# Autodesk Inventor assembly: skjellett
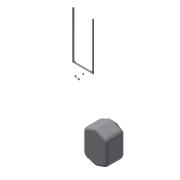
[picture p0: Inventor's stored thumbnail of the model, 180x180]
Saved by Autodesk Inventor 2014 SP1 (Build 180222100, 222)
## iProperties
Created: 2015-02-04
Part Number: skjellett
Document SubType Name: Assembly
Designer: Simen
Author: Simen
## Documents named in this file (5)
- C:\Users\Simen\Documents\git\Eit\skjellet\skjellett.iam
- main.iam
- C:\Users\Simen\Documents\git\Eit\skjellet\base.iam
- C:\Users\Simen\Documents\git\Eit\skjellet\skellett.iam
- C:\Users\Simen\Documents\git\Eit\skjellet\mount_holes_plate.ipt
## Components (3 placed, 3 different names)
1. skellett:1 [sub-assembly]
2. base:1 [sub-assembly] — Flush:1, Mate:1, Mate:2
3. mount_holes_plate:1 — Flush:1, Mate:1, Mate:2
## Relationships (3: Mate 2, Flush 1)
- Flush:1 (30 mm): base:1 ↔ mount_holes_plate:1
- Mate:1: base:1 ↔ mount_holes_plate:1
- Mate:2 (-55 mm): base:1 ↔ mount_holes_plate:1
